# Autodesk Inventor assembly: OktagonElektronik_Stage2
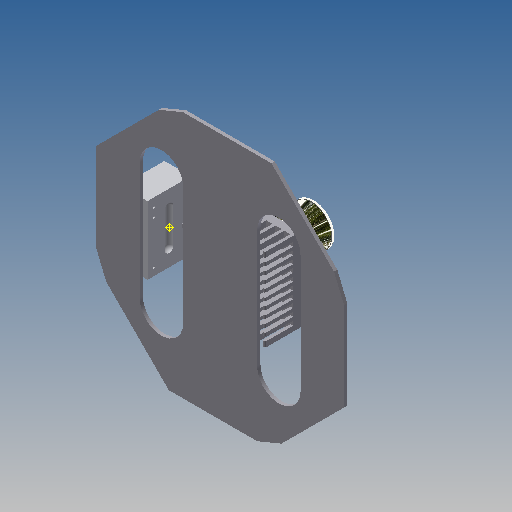
[picture p0: Inventor's stored thumbnail of the model, 512x512]
Saved by Autodesk Inventor 2018 (Build 220112000, 112)
## iProperties
Company: Fraunhofer ILT
Created: 2018-10-31
Part Number: OktagonElektronik_Stage2
Material: geeigneten Werkstoff auswählen !
Document SubType Name: Assembly
Designer: N.Grubert
Title: =Description
Author: N.Grubert
## Documents named in this file (5)
- C:\Users\knabe\Documents\GitHub\COSIMA-Laserstar\CAD\Oktokommander\OktagonElektronik_Stage2.iam
- C:\Users\knabe\Documents\GitHub\COSIMA-Laserstar\CAD\Oktokommander\Kühlkörper.ipt
- C:\Users\knabe\Documents\GitHub\COSIMA-Laserstar\CAD\Oktokommander\Stage2.ipt
- C:\Users\knabe\Documents\GitHub\COSIMA-Laserstar\CAD\Oktokommander\Parabol.ipt
- C:\Users\knabe\Documents\GitHub\COSIMA-Laserstar\CAD\Oktokommander\LDD-1000LW.ipt
## Components (7 placed, 4 different names)
1. Kühlkörper:1 — Passend:1, Passend:2, Fluchtend:1, Passend:9, Passend:10, Passend:11, Passend:12, Passend:16
2. Stage2:1 — Passend:1, Passend:2, Fluchtend:1, Passend:13, Fluchtend:6, Passend:14, Passend:15
3. Parabol:3 — Passend:3, Fluchtend:2, Passend:4, Passend:7
4. Parabol:4 — Passend:3, Fluchtend:2, Passend:4, Passend:8, Fluchtend:4, Passend:9, Winkel:1, Fluchtend:5, Passend:12
5. Parabol:5 — Passend:7, Fluchtend:4, Passend:11
6. Parabol:6 — Passend:8, Winkel:1, Fluchtend:5, Passend:10
7. LDD-1000LW:1 — Passend:13, Fluchtend:6
## Relationships (23: Mate 16, Flush 6, Angle 1)
- Passend:1 [Mate]: Kühlkörper:1 ↔ Stage2:1
- Passend:2 [Mate] (-56.5 mm): Kühlkörper:1 ↔ Stage2:1
- Fluchtend:1 [Flush] (57 mm): Kühlkörper:1 ↔ Stage2:1
- Passend:3 [Mate]: Parabol:3 ↔ Parabol:4
- Fluchtend:2 [Flush]: Parabol:3 ↔ Parabol:4
- Passend:4 [Mate] (20 mm): Parabol:3 ↔ Parabol:4
- [Mate]: Parabol:5 ↔ Parabol:6
- [Flush]: Parabol:5 ↔ Parabol:6
- [Mate] (20 mm): Parabol:5 ↔ Parabol:6
- Passend:7 [Mate] (20 mm): Parabol:3 ↔ Parabol:5
- Passend:8 [Mate] (20 mm): Parabol:4 ↔ Parabol:6
- Fluchtend:4 [Flush]: Parabol:4 ↔ Parabol:5
- Passend:9 [Mate]: Kühlkörper:1 ↔ Parabol:4
- Winkel:1 [Angle] (0 deg): Parabol:4 ↔ Parabol:6
- Fluchtend:5 [Flush]: Parabol:4 ↔ Parabol:6
- Passend:10 [Mate] (-9.1 mm): Kühlkörper:1 ↔ Parabol:6
- Passend:11 [Mate] (-9.1 mm): Kühlkörper:1 ↔ Parabol:5
- Passend:12 [Mate] (-9.1 mm): Kühlkörper:1 ↔ Parabol:4
- Passend:13 [Mate]: Stage2:1 ↔ LDD-1000LW:1
- Fluchtend:6 [Flush] (-10 mm): Stage2:1 ↔ LDD-1000LW:1
- Passend:14 [Mate]: Stage2:1
- Passend:15 [Mate]: Stage2:1
- Passend:16 [Mate]: Kühlkörper:1
## Named parameters: d6_d3 = 0 mm, d7_d4 = 0 mm, d8_d5 = 20 mm
